# Autodesk Inventor assembly: Prototype1
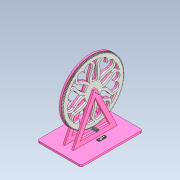
[picture p0: Inventor's stored thumbnail of the model, 180x180]
Saved by Autodesk Inventor 2021 (Build 250183000, 183)
## iProperties
Created: 2021-08-28
Part Number: Prototype1
Document SubType Name: Assembly
Designer: digge
Author: digge
## Documents named in this file (9)
- C:\Users\digge\Documents\Inventor\Projects\FerrisWheel\Prototype1.iam
- C:\Users\digge\Documents\Inventor\Projects\FerrisWheel\Base.ipt
- C:\Users\digge\Documents\Inventor\Projects\FerrisWheel\Stand.ipt
- C:\Users\digge\Documents\Inventor\Projects\FerrisWheel\Screw.ipt
- C:\Users\digge\Documents\Inventor\Projects\FerrisWheel\WheelFace.ipt
- C:\Users\digge\Documents\Inventor\Projects\FerrisWheel\WheelGear.iam
- C:\Users\digge\Documents\Inventor\Projects\FerrisWheel\MotorGear.iam
- C:\Users\digge\Documents\Inventor\Projects\FerrisWheel\Motor.ipt
- C:\Users\digge\Documents\Inventor\Projects\FerrisWheel\Arduino Nano 33 IoT.iam
## Components (9 placed, 8 different names)
1. Base:1 — Flush:1, Mate:1, Mate:2, Flush:2, Mate:3, Mate:4, Mate:11
2. Stand:1 — Flush:1, Mate:1, Mate:2, Mate:8
3. Stand:2 — Flush:2, Mate:3, Mate:4, Insert:1
4. Screw:1 — Insert:1, Mate:5, Mate:6
5. WheelFace:1 — Mate:6, Mate:7, Mate:9, Rotation:1, Mate:10, Rotation:2
6. WheelGear:1 [sub-assembly] — Mate:5, Mate:7, Mate:8, Mate:9, Rotation:1
7. MotorGear:1 [sub-assembly] — Mate:10, Rotation:2, Insert:2
8. Motor:1 — Insert:2
9. Arduino Nano 33 IoT:1 [sub-assembly] — Mate:11
## Relationships (17: Mate 11, Flush 2, Insert 2, RelateRotation 2)
- Flush:1: Base:1 ↔ Stand:1
- Mate:1: Base:1 ↔ Stand:1
- Mate:2: Base:1 ↔ Stand:1
- Flush:2: Base:1 ↔ Stand:2
- Mate:3: Base:1 ↔ Stand:2
- Mate:4: Base:1 ↔ Stand:2
- Insert:1: Stand:2 ↔ Screw:1
- Mate:5: Screw:1 ↔ WheelGear:1
- Mate:6: Screw:1 ↔ WheelFace:1
- Mate:7: WheelFace:1 ↔ WheelGear:1
- Mate:8: Stand:1 ↔ WheelGear:1
- Mate:9: WheelFace:1 ↔ WheelGear:1
- Rotation:1 [RelateRotation] (1 ul): WheelFace:1 ↔ WheelGear:1
- Mate:10: WheelFace:1 ↔ MotorGear:1
- Rotation:2 [RelateRotation] (1 ul): WheelFace:1 ↔ MotorGear:1
- Insert:2: MotorGear:1 ↔ Motor:1
- Mate:11: Base:1 ↔ Arduino Nano 33 IoT:1
